# Autodesk Inventor assembly: 810004_Power Shield ASSY
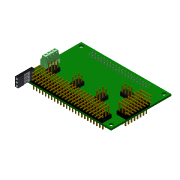
[picture p0: Inventor's stored thumbnail of the model, 180x180]
Saved by Autodesk Inventor 2015 (Build 190159000, 159)
## iProperties
Created: 2014-08-12
Part Number: 810004_Power Shield ASSY
Document SubType Name: Assembly
Designer: david
Author: david
## Documents named in this file (7)
- C:\SharedDrive\Dropbox\FAST Robotics\Products\818004_Power Shield\MECH\810004_Power Shield\810004_Power Shield ASSY.iam
- C:\SharedDrive\Dropbox\FAST Robotics\Products\810003_Radio Shield\MECH\810003_Radio Shield\810003A\702871018.ipt
- C:\SharedDrive\Dropbox\FAST Robotics\Products\818004_Power Shield\MECH\810004_Power Shield\784002_Header Right Angle 21x3 .1in.iam
- C:\SharedDrive\Dropbox\FAST Robotics\Library\784006_Phoenix 4pos .1in\MECH\784006_Phoenix 4pos .1in.iam
- C:\SharedDrive\Dropbox\FAST Robotics\Library\784001_CONN HEADER .1in SINGLE STR 40POS\CONN HEADER .1in SINGLE STR 40POS.ipt
- C:\SharedDrive\Dropbox\FAST Robotics\Products\818004_Power Shield\MECH\818002_Power Shield Bare PCB\818002A\818002A_Power Shield Bare PCB.ipt
- C:\SharedDrive\Dropbox\FAST Robotics\Library\784008_PWM Connector 1x3 .1in\Imported Components\784008_PWM Connector 1x3 .1in\Assembly1.iam
## Components (32 placed, 6 different names)
1. 818002A_Power Shield Bare PCB:1 — Mate:1, Flush:1, Flush:2, Flush:3, Flush:4, Flush:5, Mate:7, Flush:9, Flush:10, Mate:9, Mate:10, Mate:11, Mate:12, Mate:16, Mate:17, Mate:18, Mate:19, Flush:18, Flush:19, Flush:20, Flush:21, Flush:22, Flush:23, Flush:24
2. 702871018:1 — Mate:1, Flush:4, Flush:5
3. 784002_Header Right Angle 21x3 .1in:1 [sub-assembly] — Mate:15, Mate:16, Flush:18, Flush:22, Mate:20, Mate:21, Mate:22, Mate:23, Flush:25
4. 784002_Header Right Angle 21x3 .1in:3 [sub-assembly] — Mate:17, Flush:19, Mate:20, Flush:26
5. 784002_Header Right Angle 21x3 .1in:2 [sub-assembly] — Mate:18, Flush:20, Flush:23, Flush:27, Mate:24
6. 784002_Header Right Angle 21x3 .1in:5 [sub-assembly] — Mate:19, Flush:21, Flush:24, Flush:28, Mate:25
7. 784006_Phoenix 4pos .1in:1 [sub-assembly] — Mate:7, Flush:9, Flush:10
8. Assembly1:1 [sub-assembly] — Mate:15, Mate:21, Mate:22, Mate:23
9. CONN HEADER .1in SINGLE STR 40POS:7
10. CONN HEADER .1in SINGLE STR 40POS:8 — Mate:11
11. CONN HEADER .1in SINGLE STR 40POS:9
12. CONN HEADER .1in SINGLE STR 40POS:10
13. CONN HEADER .1in SINGLE STR 40POS:11 — Flush:17, Mate:24
14. CONN HEADER .1in SINGLE STR 40POS:12 — Flush:27
15. CONN HEADER .1in SINGLE STR 40POS:13 — Flush:14, Flush:26
16. CONN HEADER .1in SINGLE STR 40POS:15 — Mate:10, Flush:17
17. CONN HEADER .1in SINGLE STR 40POS:16
18. CONN HEADER .1in SINGLE STR 40POS:17
19. CONN HEADER .1in SINGLE STR 40POS:18
20. CONN HEADER .1in SINGLE STR 40POS:19
21. CONN HEADER .1in SINGLE STR 40POS:14
22. CONN HEADER .1in SINGLE STR 40POS:20 — Mate:12, Flush:28, Mate:25
23. CONN HEADER .1in SINGLE STR 40POS:21
24. CONN HEADER .1in SINGLE STR 40POS:22
25. CONN HEADER .1in SINGLE STR 40POS:23
26. CONN HEADER .1in SINGLE STR 40POS:24
27. CONN HEADER .1in SINGLE STR 40POS:1 — Flush:25
28. CONN HEADER .1in SINGLE STR 40POS:2 — Mate:9
29. CONN HEADER .1in SINGLE STR 40POS:3
30. CONN HEADER .1in SINGLE STR 40POS:4 — Flush:14
31. CONN HEADER .1in SINGLE STR 40POS:5
32. CONN HEADER .1in SINGLE STR 40POS:6
## Component patterns: (2 elements), (6 elements, first: CONN HEADER .1in SINGLE STR 40POS:7), (6 elements, first: CONN HEADER .1in SINGLE STR 40POS:13), (6 elements, first: CONN HEADER .1in SINGLE STR 40POS:14), (3 elements, first: CONN HEADER .1in SINGLE STR 40POS:1), Component Pattern 5:2 (3 elements)
## Relationships (37: Flush 20, Mate 17)
- Mate:1: 818002A_Power Shield Bare PCB:1 ↔ 702871018:1
- Flush:1: 818002A_Power Shield Bare PCB:1
- Flush:2: 818002A_Power Shield Bare PCB:1
- Flush:3: 818002A_Power Shield Bare PCB:1
- Flush:4 (-13.208 mm): 818002A_Power Shield Bare PCB:1 ↔ 702871018:1
- Flush:5 (3.048 mm): 818002A_Power Shield Bare PCB:1 ↔ 702871018:1
- Mate:7: 818002A_Power Shield Bare PCB:1 ↔ 784006_Phoenix 4pos .1in:1
- Flush:9: 818002A_Power Shield Bare PCB:1 ↔ 784006_Phoenix 4pos .1in:1
- Flush:10 (-24.13 mm): 818002A_Power Shield Bare PCB:1 ↔ 784006_Phoenix 4pos .1in:1
- Mate:9: 818002A_Power Shield Bare PCB:1 ↔ CONN HEADER .1in SINGLE STR 40POS:2
- Mate:10: 818002A_Power Shield Bare PCB:1 ↔ CONN HEADER .1in SINGLE STR 40POS:15
- Mate:11: 818002A_Power Shield Bare PCB:1 ↔ CONN HEADER .1in SINGLE STR 40POS:8
- Mate:12: 818002A_Power Shield Bare PCB:1 ↔ CONN HEADER .1in SINGLE STR 40POS:20
- Flush:14: CONN HEADER .1in SINGLE STR 40POS:13 ↔ CONN HEADER .1in SINGLE STR 40POS:4
- Flush:17: CONN HEADER .1in SINGLE STR 40POS:11 ↔ CONN HEADER .1in SINGLE STR 40POS:15
- Mate:15: 784002_Header Right Angle 21x3 .1in:1 ↔ Assembly1:1
- Mate:16: 818002A_Power Shield Bare PCB:1 ↔ 784002_Header Right Angle 21x3 .1in:1
- Mate:17: 818002A_Power Shield Bare PCB:1 ↔ 784002_Header Right Angle 21x3 .1in:3
- Mate:18: 818002A_Power Shield Bare PCB:1 ↔ 784002_Header Right Angle 21x3 .1in:2
- Mate:19: 818002A_Power Shield Bare PCB:1 ↔ 784002_Header Right Angle 21x3 .1in:5
- Flush:18: 818002A_Power Shield Bare PCB:1 ↔ 784002_Header Right Angle 21x3 .1in:1
- Flush:19: 818002A_Power Shield Bare PCB:1 ↔ 784002_Header Right Angle 21x3 .1in:3
- Flush:20: 818002A_Power Shield Bare PCB:1 ↔ 784002_Header Right Angle 21x3 .1in:2
- Flush:21: 818002A_Power Shield Bare PCB:1 ↔ 784002_Header Right Angle 21x3 .1in:5
- Flush:22 (7.62 mm): 818002A_Power Shield Bare PCB:1 ↔ 784002_Header Right Angle 21x3 .1in:1
- Flush:23 (7.62 mm): 818002A_Power Shield Bare PCB:1 ↔ 784002_Header Right Angle 21x3 .1in:2
- Mate:20 (0.127 mm): 784002_Header Right Angle 21x3 .1in:1 ↔ 784002_Header Right Angle 21x3 .1in:3
- Flush:24 (12.7 mm): 818002A_Power Shield Bare PCB:1 ↔ 784002_Header Right Angle 21x3 .1in:5
- Mate:21: 784002_Header Right Angle 21x3 .1in:1 ↔ Assembly1:1
- Mate:22: 784002_Header Right Angle 21x3 .1in:1 ↔ Assembly1:1
- Mate:23 (0.254 mm): 784002_Header Right Angle 21x3 .1in:1 ↔ Assembly1:1
- Flush:25: 784002_Header Right Angle 21x3 .1in:1 ↔ CONN HEADER .1in SINGLE STR 40POS:1
- Flush:26: 784002_Header Right Angle 21x3 .1in:3 ↔ CONN HEADER .1in SINGLE STR 40POS:13
- Flush:27: 784002_Header Right Angle 21x3 .1in:2 ↔ CONN HEADER .1in SINGLE STR 40POS:12
- Flush:28: 784002_Header Right Angle 21x3 .1in:5 ↔ CONN HEADER .1in SINGLE STR 40POS:20
- Mate:24 (5.08 mm): 784002_Header Right Angle 21x3 .1in:2 ↔ CONN HEADER .1in SINGLE STR 40POS:11
- Mate:25 (5.08 mm): 784002_Header Right Angle 21x3 .1in:5 ↔ CONN HEADER .1in SINGLE STR 40POS:20
